# Autodesk Inventor assembly: Joint Assembly
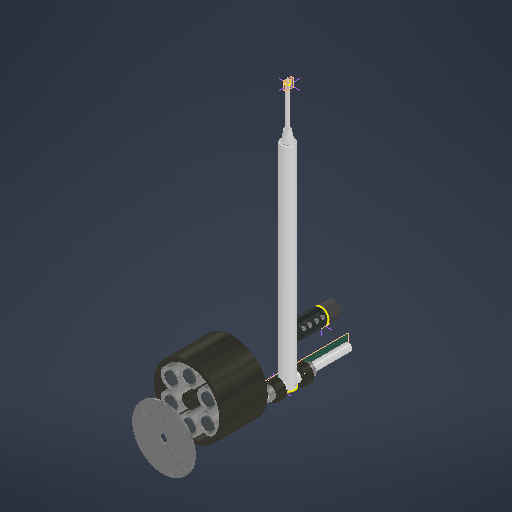
[picture p0: Inventor's stored thumbnail of the model, 512x512]
Saved by Autodesk Inventor 2026.3 (Build 303398000, 398)
## iProperties
Created: 2026-07-22
Part Number: Joint Assembly
Document SubType Name: Assembly
Designer: matot
Author: matot
## Documents named in this file (10)
- C:\Users\matot\OneDrive - Stellenbosch University\2026\MechatronicsProject478\Building the joint\Joint Assembly\Joint Assembly.iam
- C:\Users\matot\OneDrive - Stellenbosch University\2026\MechatronicsProject478\Building the joint\Joint Assembly\Brake disc.ipt
- C:\Users\matot\OneDrive - Stellenbosch University\2026\MechatronicsProject478\Building the joint\Joint Assembly\Electromagnet.iam
- C:\Users\matot\OneDrive - Stellenbosch University\2026\MechatronicsProject478\Building the joint\Joint Assembly\2058786.iam
- C:\Users\matot\OneDrive - Stellenbosch University\2026\MechatronicsProject478\Building the joint\Joint Assembly\mclx-20-20-f.iam
- C:\Users\matot\OneDrive - Stellenbosch University\2026\MechatronicsProject478\Building the joint\Joint Assembly\Reducer bushing.ipt
- C:\Users\matot\OneDrive - Stellenbosch University\2026\MechatronicsProject478\Building the joint\Joint Assembly\Optical Encoder.ipt
- C:\Users\matot\OneDrive - Stellenbosch University\2026\MechatronicsProject478\Building the joint\Joint Assembly\Rough draft shaft.ipt
- C:\Users\matot\OneDrive - Stellenbosch University\2026\MechatronicsProject478\Building the joint\Joint Assembly\8236976.ipt
- C:\Users\matot\OneDrive - Stellenbosch University\2026\MechatronicsProject478\Building the joint\Joint Assembly\Output Link.iam
## Components (11 placed, 9 different names)
1. Brake disc:1
2. Electromagnet:1 [sub-assembly]
3. 2058786:1 [sub-assembly] — Insert:11, Insert:12
4. 2058786:2 [sub-assembly] — Insert:10, Insert:13
5. mclx-20-20-f:1 [sub-assembly] — Mate:1, Insert:9
6. Reducer bushing:2 — Insert:2, Mate:1, Insert:9
7. Optical Encoder:1 — Insert:2
8. 8236976:1 — Insert:12
9. 8236976:2 — Insert:13
10. Output Link:1 [sub-assembly] — Mate:2, Mate:3, Insert:10, Insert:11
11. Rough draft shaft:1 — Mate:2, Mate:3
## Relationships (9: Insert 6, Mate 3)
- Insert:2: Reducer bushing:2 ↔ Optical Encoder:1
- Mate:1: mclx-20-20-f:1 ↔ Reducer bushing:2
- Insert:9: mclx-20-20-f:1 ↔ Reducer bushing:2
- Mate:2: Output Link:1 ↔ Rough draft shaft:1
- Mate:3: Output Link:1 ↔ Rough draft shaft:1
- Insert:10: 2058786:2 ↔ Output Link:1
- Insert:11: 2058786:1 ↔ Output Link:1
- Insert:12: 2058786:1 ↔ 8236976:1
- Insert:13: 2058786:2 ↔ 8236976:2
